# Autodesk Inventor assembly: Zespół1
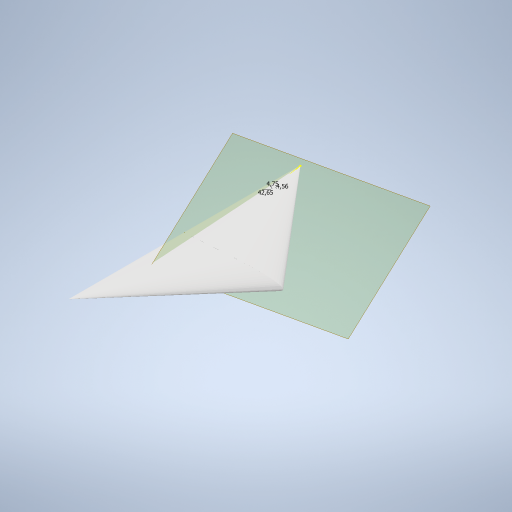
[picture p0: Inventor's stored thumbnail of the model, 512x512]
Saved by Autodesk Inventor 2023 (Build 270158000, 158)
## iProperties
Created: 2024-02-07
Part Number: Zespół1
Document SubType Name: Assembly
Designer: domin
Author: domin
## Documents named in this file (3)
- C:\Users\domin\projekty\OPIUM\fuselage\Zespół1.iam
- C:\Users\domin\projekty\OPIUM\fuselage\airfoil.ipt
- C:\Users\domin\projekty\OPIUM\fuselage\airfoil_MIR.ipt
## Components (2 placed, 2 different names)
1. airfoil:1 — Symetria:1, Zestawiające:1, Symetria:2, Symetria:3
2. airfoil_MIR:1 — Symetria:1, Zestawiające:1, Symetria:2, Symetria:3
## Relationships (4: Symmetry 3, Mate 1)
- Symetria:1 [Symmetry]: airfoil:1 ↔ airfoil_MIR:1
- Zestawiające:1 [Mate]: airfoil:1 ↔ airfoil_MIR:1
- Symetria:2 [Symmetry]: airfoil:1 ↔ airfoil_MIR:1
- Symetria:3 [Symmetry]: airfoil:1 ↔ airfoil_MIR:1
